# Autodesk Inventor assembly: Extrusion Lower Lift Stop & Switch
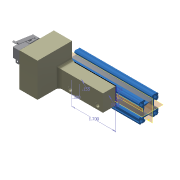
[picture p0: Inventor's stored thumbnail of the model, 180x180]
Saved by Autodesk Inventor 2018 (Build 220112000, 112)
## iProperties
Created: 2018-12-24
Part Number: Extrusion Lower Lift Stop & Switch
Document SubType Name: Assembly
Designer: ball
Author: ball
## Documents named in this file (5)
- C:\FTC\FTC8863CAD\2018Robot\Extrusion Lower Lift Stop & Switch.iam
- C:\FTC\FTC8863CAD\Actobotics\565 parts\565018.ipt
- C:\FTC\FTC8863CAD\Actobotics\585 parts\585718.ipt
- C:\FTC\FTC8863CAD\2018Robot\Lower Lift Limit & Stop.ipt
- C:\FTC\FTC8863CAD\Actobotics\605 parts\605632.ipt
## Components (4 placed, 4 different names)
1. 565018:1 — Mate:1, Mate:2, Flush:1, Flush:2
2. 585718:1 — Mate:1, Mate:2
3. Lower Lift Limit & Stop:1 — Flush:1, Flush:2, Flush:3, Mate:3, Flush:4
4. 605632:2 — Flush:3, Mate:3, Flush:4
## Relationships (7: Flush 4, Mate 3)
- Mate:1: 565018:1 ↔ 585718:1
- Mate:2: 565018:1 ↔ 585718:1
- Flush:1: 565018:1 ↔ Lower Lift Limit & Stop:1
- Flush:2: 565018:1 ↔ Lower Lift Limit & Stop:1
- Flush:3: Lower Lift Limit & Stop:1 ↔ 605632:2
- Mate:3: Lower Lift Limit & Stop:1 ↔ 605632:2
- Flush:4: Lower Lift Limit & Stop:1 ↔ 605632:2
